# Autodesk Inventor assembly: cnc_plate
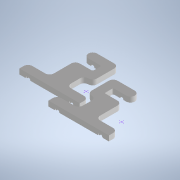
[picture p0: Inventor's stored thumbnail of the model, 180x180]
Saved by Autodesk Inventor 2020 (Build 240168000, 168)
## iProperties
Created: 2020-03-17
Part Number: cnc_plate
Document SubType Name: Assembly
Designer: erwin
Author: erwin
## Documents named in this file (3)
- D:\GitHub\BeachMaid\platform-2\trailer\cnc_plate.iam
- D:\GitHub\BeachMaid\platform-2\trailer\clamp.ipt
- D:\GitHub\BeachMaid\platform-2\trailer\clamp_MIR.ipt
## Components (2 placed, 2 different names)
1. clamp:1 — Flush:1
2. clamp_MIR:1 — Flush:1
## Relationships (1: Flush 1)
- Flush:1: clamp:1 ↔ clamp_MIR:1
